# Autodesk Inventor assembly: CanBusHolder
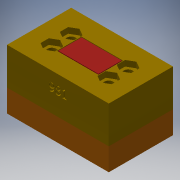
[picture p0: Inventor's stored thumbnail of the model, 180x180]
Saved by Autodesk Inventor 2018.1 (Build 221171000, 171)
## iProperties
Created: 2017-10-25
Part Number: CanBusHolder
Document SubType Name: Assembly
Designer: steele
Author: steele
## Documents named in this file (4)
- D:\snobotics\CAD-Development\robSteele\2018RobotParts\CanBusHolder.iam
- D:\snobotics\CAD-Development\robSteele\2018RobotParts\BaseForCanBusConnector.ipt
- D:\snobotics\CAD-Development\robSteele\2018RobotParts\canConnectorModel.ipt
- D:\snobotics\CAD-Development\robSteele\2018RobotParts\CapForCanBusConnector.ipt
## Components (3 placed, 3 different names)
1. BaseForCanBusConnector:1 — Mate:1, Flush:1, Flush:2, Mate:2
2. canConnectorModel:1 — Mate:1, Flush:1, Flush:2, Flush:3, Flush:4
3. CapForCanBusConnector:1 — Mate:2, Flush:3, Flush:4
## Relationships (6: Flush 4, Mate 2)
- Mate:1: BaseForCanBusConnector:1 ↔ canConnectorModel:1
- Flush:1: BaseForCanBusConnector:1 ↔ canConnectorModel:1
- Flush:2: BaseForCanBusConnector:1 ↔ canConnectorModel:1
- Mate:2: BaseForCanBusConnector:1 ↔ CapForCanBusConnector:1
- Flush:3: canConnectorModel:1 ↔ CapForCanBusConnector:1
- Flush:4: canConnectorModel:1 ↔ CapForCanBusConnector:1
